# Autodesk Inventor assembly: maquette
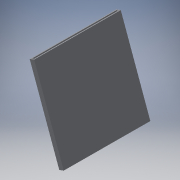
[picture p0: Inventor's stored thumbnail of the model, 180x180]
Saved by Autodesk Inventor 2017 (Build 210142000, 142)
## iProperties
Created: 2017-03-06
Part Number: maquette
Document SubType Name: Assembly
Designer: LaFaucheuse
Author: LaFaucheuse
## Documents named in this file (4)
- D:\[DATA]\[SW]\projetLDB\maquette.iam
- D:\[DATA]\[SW]\projetLDB\cote.ipt
- D:\[DATA]\[SW]\projetLDB\face.ipt
- face.ipt
## Components (4 placed, 2 different names)
1. cote:1 — Placage:2, Placage:3, Placage:7, Placage:8
2. cote:2 — Placage:1, Placage:4, Placage:5, Placage:6
3. face:1 — Placage:1, Placage:2, Placage:3, Placage:4
4. face:2 — Placage:5, Placage:6, Placage:7, Placage:8
## Relationships (8: Mate 8)
- Placage:1 [Mate]: cote:2 ↔ face:1
- Placage:2 [Mate]: cote:1 ↔ face:1
- Placage:3 [Mate]: cote:1 ↔ face:1
- Placage:4 [Mate]: cote:2 ↔ face:1
- Placage:5 [Mate]: cote:2 ↔ face:2
- Placage:6 [Mate]: cote:2 ↔ face:2
- Placage:7 [Mate]: cote:1 ↔ face:2
- Placage:8 [Mate]: cote:1 ↔ face:2
